# Autodesk Inventor assembly: Assembly
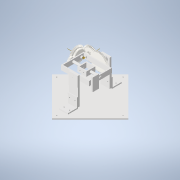
[picture p0: Inventor's stored thumbnail of the model, 180x180]
Saved by Autodesk Inventor 2022 (Build 260153000, 153)
## iProperties
Created: 2023-02-01
Part Number: Assembly
Document SubType Name: Assembly
Designer: Deven Joshi
Author: Deven Joshi
## Documents named in this file (12)
- C:\Users\ac_jo\OneDrive\Documents\TA202\Assembly.iam
- C:\Users\ac_jo\OneDrive\Documents\TA202\Frame.ipt
- C:\Users\ac_jo\OneDrive\Documents\TA202\Assembly\Design Accelerator\Bevel Gears1.iam
- C:\Users\ac_jo\OneDrive\Documents\Labta202\Part4.ipt
- C:\Users\ac_jo\OneDrive\Documents\TA202\Assembly\Design Accelerator\Spur Gears1.iam
- C:\Users\ac_jo\OneDrive\Documents\TA202\Assembly\Design Accelerator\Spur Gears2.iam
- C:\Users\ac_jo\OneDrive\Documents\TA202\Assembly\Design Accelerator\Spur Gears5.iam
- C:\Users\ac_jo\OneDrive\Documents\TA202\Angle.ipt
- C:\Users\ac_jo\OneDrive\Documents\TA202\Stand.ipt
- C:\Users\ac_jo\OneDrive\Documents\TA202\Base Plate.ipt
- C:\Users\ac_jo\OneDrive\Documents\TA202\SpurFixed.iam
- C:\Users\ac_jo\OneDrive\Documents\TA202\CounterWeight.ipt
## Components (19 placed, 9 different names)
1. Frame:1 — Mate:7, Mate:8, Mate:12, Mate:16, Mate:17, Mate:18, Mate:19, Mate:20, Mate:21, Mate:31, Mate:33, Mate:36, Mate:43, Mate:45, Mate:49, Angle:1
2. Bevel Gears:1 [sub-assembly] — Mate:45, Mate:46, Mate:47
3. Part4:1 — Mate:46
4. Part4:2 — Mate:12, Mate:15
5. Part4:3 — Mate:5, Mate:43, Mate:47
6. Spur Gears:2 [sub-assembly] — Mate:5, Mate:17
7. Spur Gears:3 [sub-assembly] — Mate:7, Mate:8
8. Spur Gears:4 [sub-assembly]
9. Spur Gears:5 [sub-assembly] — Mate:15, Mate:16, Mate:48
10. Angle:1 — Mate:25, Mate:26, Mate:27
11. Stand:1 — Mate:18, Mate:19, Mate:22, Mate:23, Mate:24, Mate:37
12. Stand:2 — Mate:20, Mate:21, Mate:25, Mate:26, Mate:27
13. Angle:2 — Mate:22, Mate:23, Mate:24, Mate:28, Mate:29, Mate:30
14. Base Plate:1 — Mate:28, Mate:29, Mate:30
15. Part4:4 — Mate:31
16. Part4:5 — Mate:33
17. SpurFixed:1 [sub-assembly] — Mate:36, Mate:37
18. Part4:6 — Mate:48
19. CounterWeight:1 — Mate:49, Angle:1
## Relationships (31: Mate 30, Angle 1)
- Mate:5: Part4:3 ↔ Spur Gears:2
- Mate:7: Frame:1 ↔ Spur Gears:3
- Mate:8 (3 mm): Frame:1 ↔ Spur Gears:3
- Mate:12: Frame:1 ↔ Part4:2
- Mate:15: Part4:2 ↔ Spur Gears:5
- Mate:16 (3 mm): Frame:1 ↔ Spur Gears:5
- Mate:17 (3 mm): Frame:1 ↔ Spur Gears:2
- Mate:18: Frame:1 ↔ Stand:1
- Mate:19: Frame:1 ↔ Stand:1
- Mate:20: Frame:1 ↔ Stand:2
- Mate:21: Frame:1 ↔ Stand:2
- Mate:22: Stand:1 ↔ Angle:2
- Mate:23: Stand:1 ↔ Angle:2
- Mate:24: Stand:1 ↔ Angle:2
- Mate:25: Angle:1 ↔ Stand:2
- Mate:26: Angle:1 ↔ Stand:2
- Mate:27: Angle:1 ↔ Stand:2
- Mate:28: Angle:2 ↔ Base Plate:1
- Mate:29: Angle:2 ↔ Base Plate:1
- Mate:30: Angle:2 ↔ Base Plate:1
- Mate:31: Frame:1 ↔ Part4:4
- Mate:33: Frame:1 ↔ Part4:5
- Mate:36: Frame:1 ↔ SpurFixed:1
- Mate:37: Stand:1 ↔ SpurFixed:1
- Mate:43: Frame:1 ↔ Part4:3
- Mate:45: Frame:1 ↔ Bevel Gears:1
- Mate:46: Bevel Gears:1 ↔ Part4:1
- Mate:47: Bevel Gears:1 ↔ Part4:3
- Mate:48: Spur Gears:5 ↔ Part4:6
- Mate:49: Frame:1 ↔ CounterWeight:1
- Angle:1 (0 deg): Frame:1 ↔ CounterWeight:1
